# Autodesk Inventor assembly: Assembly1
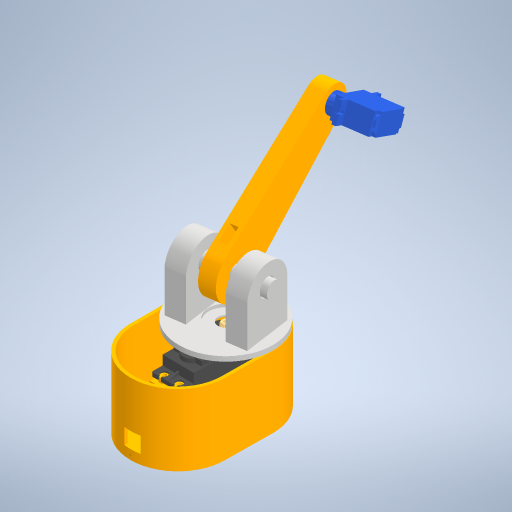
[picture p0: Inventor's stored thumbnail of the model, 512x512]
Saved by Autodesk Inventor 2024 (Build 280153000, 153)
## iProperties
Created: 2024-04-28
Part Number: Assembly1
Document SubType Name: Assembly
Designer: samue
Author: samue
## Documents named in this file (8)
- D:\samue\Escritorio\OneDrive - UVG\UVG\Año 2024\Semestre 1\Progra micros\Practicas\Brazo_robotico\Diseños 3D\Assembly1.iam
- D:\samue\Escritorio\OneDrive - UVG\UVG\Año 2024\Semestre 1\Progra micros\Practicas\Brazo_robotico\Diseños 3D\Servo SG90\Servo SG90.ipt
- D:\samue\Escritorio\OneDrive - UVG\UVG\Año 2024\Semestre 1\Progra micros\Practicas\Brazo_robotico\Diseños 3D\eje de motor.ipt
- D:\samue\Escritorio\OneDrive - UVG\UVG\Año 2024\Semestre 1\Progra micros\Practicas\Brazo_robotico\Diseños 3D\Brazo.ipt
- D:\samue\Escritorio\OneDrive - UVG\UVG\Año 2024\Semestre 1\Progra micros\Practicas\Brazo_robotico\Diseños 3D\EJE BRAZO.ipt
- D:\samue\Escritorio\OneDrive - UVG\UVG\Año 2024\Semestre 1\Progra micros\Practicas\Brazo_robotico\Diseños 3D\MG995\MG995.ipt
- D:\samue\Escritorio\OneDrive - UVG\UVG\Año 2024\Semestre 1\Progra micros\Practicas\Brazo_robotico\Diseños 3D\Base.ipt
- D:\samue\Escritorio\OneDrive - UVG\UVG\Año 2024\Semestre 1\Progra micros\Practicas\Brazo_robotico\Diseños 3D\base2.ipt
## Components (7 placed, 7 different names)
1. Servo SG90:1 — Rotational:1
2. eje de motor:1 — Rotational:1, Mate:1, Mate:2
3. Brazo:1 — Mate:1, Mate:2, Cylindrical:1
4. EJE BRAZO:1 — Cylindrical:1, Mate:5
5. MG995:1 — Rigid:1
6. base2:1 — Mate:3, Mate:4, Rigid:1, Mate:5
7. Base:1 — Mate:3, Mate:4
## Relationships (8: Mate 5, RevoluteJoint 1, CylindricalJoint 1, WeldJoint 1)
- Rotational:1 [RevoluteJoint] (1 mm): Servo SG90:1 ↔ eje de motor:1
- Mate:1: eje de motor:1 ↔ Brazo:1
- Mate:2: eje de motor:1 ↔ Brazo:1
- Cylindrical:1: Brazo:1 ↔ EJE BRAZO:1
- Mate:3: base2:1 ↔ Base:1
- Mate:4: base2:1 ↔ Base:1
- Rigid:1 [WeldJoint]: MG995:1 ↔ base2:1
- Mate:5: EJE BRAZO:1 ↔ base2:1
